# Autodesk Inventor assembly: structure_channel_mirrored
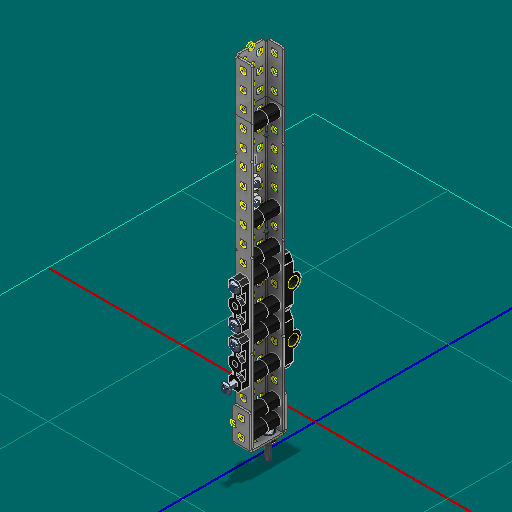
[picture p0: Inventor's stored thumbnail of the model, 512x512]
Saved by Autodesk Inventor 2025 (Build 290162000, 162)
## iProperties
Created: 2024-08-18
Part Number: structure_channel_mirrored
Document SubType Name: Assembly
Designer: averey
Author: averey
## Documents named in this file (19)
- C:\Users\avere\vex_robotics_high_stakes\hardware\cad\ATLAS\tower\structure\structure_half_mirrored\structure_channel_mirrored.iam
- C:\Users\avere\vex_robotics_high_stakes\hardware\cad\ATLAS\tower\structure\structure_half_mirrored\Alu C 1x2x1x20_mirrored.ipt
- C:\Users\avere\vex_robotics_high_stakes\hardware\cad\ATLAS\tower\structure\structure_half_mirrored\Alu C 2x2x2x1_mirrored.ipt
- C:\Users\avere\vex_robotics_high_stakes\hardware\cad\VEX-CAD-Inventor\Motion\Spacers\Spacer Nylon .375 OD\NSpacer .375 OD x .375.ipt
- C:\Users\avere\vex_robotics_high_stakes\hardware\cad\VEX-CAD-Inventor\Motion\Spacers\Spacer Nylon .375 OD.ipt
- C:\Users\avere\vex_robotics_high_stakes\hardware\cad\VEX-CAD-Inventor\Motion\Spacers\Spacer Nylon .375 OD\NSpacer .375 OD x .500.ipt
- C:\Users\avere\vex_robotics_high_stakes\hardware\cad\ATLAS\tower\structure\structure_half_mirrored\Alu C 1x2x1x17_mirrored.ipt
- C:\Users\avere\vex_robotics_high_stakes\hardware\cad\VEX-CAD-Inventor\Motion\Spacers\Spacer Nylon .375 OD\NSpacer .375 OD x .125.ipt
- C:\Users\avere\vex_robotics_high_stakes\hardware\cad\VEX-CAD-Inventor\Motion\Spacers\Washer Steel\SWasher .375 OD x .015625.ipt
- C:\Users\avere\vex_robotics_high_stakes\hardware\cad\VEX-CAD-Inventor\Motion\Spacers\Washer Steel.ipt
- C:\Users\avere\vex_robotics_high_stakes\hardware\cad\VEX-CAD-Inventor\Motion\Spacers\Washer Steel\SWasher .375 OD x .031250.ipt
- C:\Users\avere\vex_robotics_high_stakes\hardware\cad\VEX-CAD-Inventor\Structure\Hardware\Screw Steel - Star\SScrew Star Smooth .750.ipt
- C:\Users\avere\vex_robotics_high_stakes\hardware\cad\VEX-CAD-Inventor\Structure\Hardware\Screw Steel - Star.ipt
- C:\Users\avere\vex_robotics_high_stakes\hardware\cad\ATLAS\tower\structure\structure_half_mirrored\HS Pillow Bearing Block_mirrored.ipt
- C:\Users\avere\vex_robotics_high_stakes\hardware\cad\ATLAS\tower\structure\structure_half_mirrored\Bearing Flat_mirrored.ipt
- C:\Users\avere\vex_robotics_high_stakes\hardware\cad\VEX-CAD-Inventor\Structure\Hardware\Screw Steel - Star\SScrew Star Smooth 1.500.ipt
- C:\Users\avere\vex_robotics_high_stakes\hardware\cad\ATLAS\tower\structure\structure_half_mirrored\Nut Thin Nylock_mirrored.ipt
- C:\Users\avere\vex_robotics_high_stakes\hardware\cad\ATLAS\tower\structure\structure_half_mirrored\bearing_flat_w_hardware_offset_mirrored.iam
- C:\Users\avere\vex_robotics_high_stakes\hardware\cad\VEX-CAD-Inventor\Structure\Hardware\Screw Steel - Star\SScrew Star Smooth 1.750.ipt
## Components (38 placed, 15 different names)
1. Alu C 1x2x1x20_mirrored:1 — Mate:5, Angle:2, Angle:1, Mate:6, Insert:1, Insert:3, Insert:5, Mate:7, Insert:6
2. Alu C 2x2x2x1_mirrored:1 — Mate:6, Insert:1, Insert:9, Insert:10
3. NSpacer .375 OD x .375:1 — Insert:2
4. NSpacer .375 OD x .500:2 — Insert:3, Insert:2
5. NSpacer .375 OD x .375:3 — Insert:4
6. NSpacer .375 OD x .500:4 — Insert:5, Insert:4
7. Alu C 1x2x1x17_mirrored:1 — Mate:7, Insert:6, Mate:12, Insert:15, Mate:13, Insert:16, Insert:18, Insert:20, Insert:22, Insert:24, Mate:14, Insert:25, Mate:15, Insert:26, Insert:39, Insert:37, Insert:41, Insert:40, Mate:10
8. NSpacer .375 OD x .125:5 — Insert:9, Insert:8
9. SWasher .375 OD x .015625:1 — Insert:7
10. SWasher .375 OD x .031250:2 — Insert:8, Insert:7
11. SScrew Star Smooth .750:1 — Insert:10
12. HS Pillow Bearing Block_mirrored:1 — Mate:12, Insert:15, Insert:32, Insert:31
13. HS Pillow Bearing Block_mirrored:2 — Mate:13, Insert:16, Insert:34, Insert:33
14. NSpacer .375 OD x .375:6 — Insert:17
15. NSpacer .375 OD x .500:7 — Insert:18, Insert:17
16. NSpacer .375 OD x .375:8 — Insert:19
17. NSpacer .375 OD x .500:9 — Insert:20, Insert:19
18. NSpacer .375 OD x .375:10 — Insert:21
19. NSpacer .375 OD x .500:11 — Insert:22, Insert:21
20. NSpacer .375 OD x .375:12 — Insert:23
21. NSpacer .375 OD x .500:13 — Insert:24, Insert:23
22. Bearing Flat_mirrored:1 — Mate:14, Insert:25, Insert:29, Insert:42
23. Bearing Flat_mirrored:2 — Mate:15, Insert:26, Insert:27, Insert:28
24. SScrew Star Smooth 1.500:2 — Insert:27
25. SScrew Star Smooth 1.500:3 — Insert:28
26. SScrew Star Smooth 1.500:4 — Insert:29
27. Nut Thin Nylock_mirrored:1 — Insert:34
28. Nut Thin Nylock_mirrored:2 — Insert:32
29. Nut Thin Nylock_mirrored:3 — Insert:33
30. Nut Thin Nylock_mirrored:4 — Insert:31
31. bearing_flat_w_hardware_offset_mirrored:1 [sub-assembly] — Insert:40, Mate:10
32. NSpacer .375 OD x .375:14 — Insert:38
33. NSpacer .375 OD x .500:15 — Insert:39, Insert:38
34. NSpacer .375 OD x .375:16 — Insert:36
35. NSpacer .375 OD x .500:17 — Insert:37, Insert:36
36. NSpacer .375 OD x .375:18 — Insert:40
37. NSpacer .375 OD x .500:19 — Insert:41, Insert:40
38. SScrew Star Smooth 1.750:5 — Insert:42
## Relationships (47: Insert 37, Mate 8, Angle 2)
- Mate:5 (49.6316 mm): Alu C 1x2x1x20_mirrored:1
- Angle:2 (0 deg): Alu C 1x2x1x20_mirrored:1
- Angle:1 (0 deg): Alu C 1x2x1x20_mirrored:1
- Mate:6: Alu C 1x2x1x20_mirrored:1 ↔ Alu C 2x2x2x1_mirrored:1
- Insert:1: Alu C 1x2x1x20_mirrored:1 ↔ Alu C 2x2x2x1_mirrored:1
- Insert:3: Alu C 1x2x1x20_mirrored:1 ↔ NSpacer .375 OD x .500:2
- Insert:2: NSpacer .375 OD x .375:1 ↔ NSpacer .375 OD x .500:2
- Insert:5: Alu C 1x2x1x20_mirrored:1 ↔ NSpacer .375 OD x .500:4
- Insert:4: NSpacer .375 OD x .375:3 ↔ NSpacer .375 OD x .500:4
- Mate:7: Alu C 1x2x1x20_mirrored:1 ↔ Alu C 1x2x1x17_mirrored:1
- Insert:6: Alu C 1x2x1x20_mirrored:1 ↔ Alu C 1x2x1x17_mirrored:1
- Insert:9: Alu C 2x2x2x1_mirrored:1 ↔ NSpacer .375 OD x .125:5
- Insert:8: NSpacer .375 OD x .125:5 ↔ SWasher .375 OD x .031250:2
- Insert:7: SWasher .375 OD x .015625:1 ↔ SWasher .375 OD x .031250:2
- Insert:10: Alu C 2x2x2x1_mirrored:1 ↔ SScrew Star Smooth .750:1
- Mate:12: Alu C 1x2x1x17_mirrored:1 ↔ HS Pillow Bearing Block_mirrored:1
- Insert:15: Alu C 1x2x1x17_mirrored:1 ↔ HS Pillow Bearing Block_mirrored:1
- Mate:13: Alu C 1x2x1x17_mirrored:1 ↔ HS Pillow Bearing Block_mirrored:2
- Insert:16: Alu C 1x2x1x17_mirrored:1 ↔ HS Pillow Bearing Block_mirrored:2
- Insert:18: Alu C 1x2x1x17_mirrored:1 ↔ NSpacer .375 OD x .500:7
- Insert:17: NSpacer .375 OD x .375:6 ↔ NSpacer .375 OD x .500:7
- Insert:20: Alu C 1x2x1x17_mirrored:1 ↔ NSpacer .375 OD x .500:9
- Insert:19: NSpacer .375 OD x .375:8 ↔ NSpacer .375 OD x .500:9
- Insert:22: Alu C 1x2x1x17_mirrored:1 ↔ NSpacer .375 OD x .500:11
- Insert:21: NSpacer .375 OD x .375:10 ↔ NSpacer .375 OD x .500:11
- Insert:24: Alu C 1x2x1x17_mirrored:1 ↔ NSpacer .375 OD x .500:13
- Insert:23: NSpacer .375 OD x .375:12 ↔ NSpacer .375 OD x .500:13
- Mate:14: Alu C 1x2x1x17_mirrored:1 ↔ Bearing Flat_mirrored:1
- Insert:25: Alu C 1x2x1x17_mirrored:1 ↔ Bearing Flat_mirrored:1
- Mate:15: Alu C 1x2x1x17_mirrored:1 ↔ Bearing Flat_mirrored:2
- Insert:26: Alu C 1x2x1x17_mirrored:1 ↔ Bearing Flat_mirrored:2
- Insert:27: Bearing Flat_mirrored:2 ↔ SScrew Star Smooth 1.500:2
- Insert:28: Bearing Flat_mirrored:2 ↔ SScrew Star Smooth 1.500:3
- Insert:29: Bearing Flat_mirrored:1 ↔ SScrew Star Smooth 1.500:4
- Insert:34: HS Pillow Bearing Block_mirrored:2 ↔ Nut Thin Nylock_mirrored:1
- Insert:32: HS Pillow Bearing Block_mirrored:1 ↔ Nut Thin Nylock_mirrored:2
- Insert:33: HS Pillow Bearing Block_mirrored:2 ↔ Nut Thin Nylock_mirrored:3
- Insert:31: HS Pillow Bearing Block_mirrored:1 ↔ Nut Thin Nylock_mirrored:4
- Insert:39: Alu C 1x2x1x17_mirrored:1 ↔ NSpacer .375 OD x .500:15
- Insert:38: NSpacer .375 OD x .375:14 ↔ NSpacer .375 OD x .500:15
- Insert:37: Alu C 1x2x1x17_mirrored:1 ↔ NSpacer .375 OD x .500:17
- Insert:36: NSpacer .375 OD x .375:16 ↔ NSpacer .375 OD x .500:17
- Insert:41: Alu C 1x2x1x17_mirrored:1 ↔ NSpacer .375 OD x .500:19
- Insert:40: NSpacer .375 OD x .375:18 ↔ NSpacer .375 OD x .500:19
- Insert:42 (6.35 mm): Bearing Flat_mirrored:1 ↔ SScrew Star Smooth 1.750:5
- Insert:40: Alu C 1x2x1x17_mirrored:1 ↔ bearing_flat_w_hardware_offset_mirrored:1
- Mate:10: Alu C 1x2x1x17_mirrored:1 ↔ bearing_flat_w_hardware_offset_mirrored:1
